# Autodesk Inventor assembly: gu1e_round-round
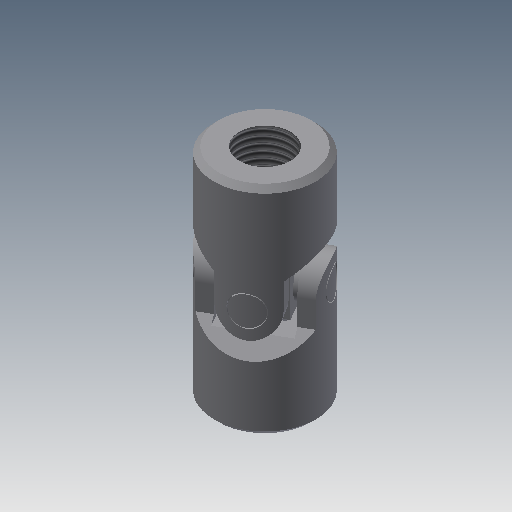
[picture p0: Inventor's stored thumbnail of the model, 512x512]
Saved by Autodesk Inventor 2021 (Build 250183000, 183)
## iProperties
Company: TraceParts S.A.
Created: 2021-03-16
Part Number: gu1e_round-round
Checked By: TraceParts S.A.
Catalog Web Link: www.traceparts.com
Document SubType Name: Assembly
Designer: TraceParts
Mass: 42.3963 g
Surface Area: 144.632 cm^2
Volume: 42.3963 cm^3
Density: 1 g/cm^3
DESIGN: GUE cardanic DIN808
SUPPLIER: SIT
TraceParts.PartNumber: 32-28022007-067680
TraceParts.PartTitle: GUE cardanic DIN808
TraceParts.InstanceId: 32-28022007-067680JHA2HX92DB50YX739C172EFG
TraceParts.PartStatus: Published
TraceParts.PartVersion: 1.1.7
TRACEPARTS: TRACEPARTS
TraceParts.PartLanguage: en
TraceParts.ClassPath: SIT:32-28022007-067680
Author: TraceParts
## Documents named in this file (4)
- C:\Users\Santiago Suárez\Documents\GitHub\Dis.-Mecatronico-E6\inventor proyecto\Cardan\cardan.iam
- C:\Users\Santiago Suárez\Documents\GitHub\Dis.-Mecatronico-E6\inventor proyecto\Cardan\gu1e_round-round_01.ipt
- C:\Users\Santiago Suárez\Documents\GitHub\Dis.-Mecatronico-E6\inventor proyecto\Cardan\gu1e_round-round_02.ipt
- C:\Users\Santiago Suárez\Documents\GitHub\Dis.-Mecatronico-E6\inventor proyecto\Cardan\gu1e_round-round_03.ipt
## Components (3 placed, 3 different names)
1. gu1e_round-round_01:1 — Rotational:3, Mate:1
2. gu1e_round-round_02:1 — Rotational:2
3. gu1e_round-round_03:1 — Rotational:2, Rotational:3
## Relationships (3: RevoluteJoint 2, Mate 1)
- Rotational:2 [RevoluteJoint]: gu1e_round-round_02:1 ↔ gu1e_round-round_03:1
- Rotational:3 [RevoluteJoint]: gu1e_round-round_01:1 ↔ gu1e_round-round_03:1
- Mate:1: gu1e_round-round_01:1
